# Autodesk Inventor assembly: Ponte Menor Assembly
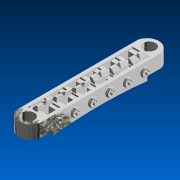
[picture p0: Inventor's stored thumbnail of the model, 180x180]
Saved by Autodesk Inventor 2016 (Build 200138000, 138)
## iProperties
Created: 2018-12-10
Part Number: Ponte Menor Assembly
Document SubType Name: Assembly
Designer: lesly
Author: lesly
## Documents named in this file (4)
- C:\Users\lesly\Desktop\Projeto CAD Eng Mecânica\Ponte Menor Assembly.iam
- C:\Users\lesly\Desktop\Projeto CAD Eng Mecânica\Ponte menor.ipt
- C:\Users\lesly\Desktop\Projeto CAD Eng Mecânica\parafuso interno da ponte.ipt
- C:\Users\lesly\Desktop\Projeto CAD Eng Mecânica\Apoio móvel da ponte.ipt
## Components (13 placed, 3 different names)
1. Ponte menor:2 — Insert:1, Insert:2, Insert:3, Insert:4, Insert:5, Insert:6, Insert:7, Insert:8, Insert:9, Insert:10, Insert:11, Insert:12
2. parafuso interno da ponte:1 — Insert:1
3. parafuso interno da ponte:2 — Insert:6
4. parafuso interno da ponte:3 — Insert:5
5. parafuso interno da ponte:4 — Insert:4
6. parafuso interno da ponte:5 — Insert:3
7. parafuso interno da ponte:6 — Insert:2
8. Apoio móvel da ponte:1 — Insert:7
9. Apoio móvel da ponte:2 — Insert:8
10. Apoio móvel da ponte:3 — Insert:9
11. Apoio móvel da ponte:4 — Insert:10
12. Apoio móvel da ponte:5 — Insert:11
13. Apoio móvel da ponte:6 — Insert:12
## Relationships (12: Insert 12)
- Insert:1: Ponte menor:2 ↔ parafuso interno da ponte:1
- Insert:2: Ponte menor:2 ↔ parafuso interno da ponte:6
- Insert:3: Ponte menor:2 ↔ parafuso interno da ponte:5
- Insert:4: Ponte menor:2 ↔ parafuso interno da ponte:4
- Insert:5: Ponte menor:2 ↔ parafuso interno da ponte:3
- Insert:6: Ponte menor:2 ↔ parafuso interno da ponte:2
- Insert:7: Ponte menor:2 ↔ Apoio móvel da ponte:1
- Insert:8 (1 mm): Ponte menor:2 ↔ Apoio móvel da ponte:2
- Insert:9 (2 mm): Ponte menor:2 ↔ Apoio móvel da ponte:3
- Insert:10 (3 mm): Ponte menor:2 ↔ Apoio móvel da ponte:4
- Insert:11 (4 mm): Ponte menor:2 ↔ Apoio móvel da ponte:5
- Insert:12 (5 mm): Ponte menor:2 ↔ Apoio móvel da ponte:6
